# Autodesk Inventor assembly: ЛЦМК000002.00.03.00.00.00 Облегченный вариант крепления
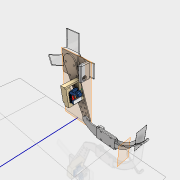
[picture p0: Inventor's stored thumbnail of the model, 180x180]
Saved by Autodesk Inventor 2021.2 (Build 252289000, 289)
## iProperties
Created: 2025-11-11
Part Number: ЛЦМК000002.00.03.00.00.00 Облегченный вариант крепления
Document SubType Name: Assembly
Designer: Захаров
Author: Захаров
## Documents named in this file (12)
- C:\Users\User\Documents\CaseARHead1\ЛЦМК000002.00.03.00.00.00 Облегченный вариант крепления.iam
- ЛЦМК000002.00.03.00.00.00 Облегченный вариант крепления.iam
- C:\Users\User\Documents\CaseARHead1\ЛЦМК000002.00.00.00.00.08-01.ipt
- C:\Users\User\Documents\CaseARHead1\ЛЦМК000002.00.00.00.00.15.ipt
- C:\Users\User\Documents\CaseARHead1\ЛЦМК000002.00.00.00.00.18-01.ipt
- C:\Users\User\Documents\CaseARHead1\ЛЦМК000002.00.00.00.00.19 мост.ipt
- C:\Users\User\Documents\CaseARHead1\ЛЦМК000002.00.00.00.00.06-10.ipt
- C:\Users\User\Documents\CaseARHead1\Сборка1.iam
- C:\Users\User\Documents\Inventor\Content Center Files\R2021\ru-RU\Screw A2 GOST 17473-80\Винт A2.M3-6gx6 ГОСТ 17473-80.ipt
- C:\Users\User\Documents\CaseARHead1\ЛЦМК000002.00.00.00.00.20 Платформа экрана.ipt
- C:\Users\User\Documents\CaseARHead1\ЛЦМК000002.00.00.00.00.13 OLED.ipt
- C:\Users\User\Documents\CaseARHead1\ЛЦМК000002.00.00.00.00.14 Фиксатор OLED.ipt
## Components (10 placed, 10 different names)
1. ЛЦМК000002.00.00.00.00.08-01:1 — Вставка:1, Вставка:2
2. ЛЦМК000002.00.00.00.00.15:1 — Вставка:1, Вставка:2, Заподлицо:1, Совмещение:1, Заподлицо:2
3. ЛЦМК000002.00.00.00.00.18-01:1 — Заподлицо:1, Совмещение:1, Заподлицо:2, Вставка:3, Вставка:4
4. ЛЦМК000002.00.00.00.00.19 мост:1 — Вставка:3, Вставка:4, Совмещение:2, Вставка:5, Заподлицо:3, Заподлицо:4
5. ЛЦМК000002.00.00.00.00.06-10:1 — Совмещение:2, Вставка:5, Совмещение:3, Совмещение:4
6. Сборка1:1 [sub-assembly] — Совмещение:3, Совмещение:4
7. Винт A2 ГОСТ 17473-80 M3-6gx6:1
8. ЛЦМК000002.00.00.00.00.20 Платформа экрана:1 — Заподлицо:3, Заподлицо:4, Вставка:6, Вставка:7, Вставка:8, Вставка:9
9. ЛЦМК000002.00.00.00.00.13 OLED:1 — Вставка:6, Вставка:7
10. ЛЦМК000002.00.00.00.00.14 Фиксатор OLED:1 — Вставка:8, Вставка:9
## Relationships (17: Insert 9, Flush 4, Mate 4)
- Вставка:1 [Insert]: ЛЦМК000002.00.00.00.00.08-01:1 ↔ ЛЦМК000002.00.00.00.00.15:1
- Вставка:2 [Insert]: ЛЦМК000002.00.00.00.00.08-01:1 ↔ ЛЦМК000002.00.00.00.00.15:1
- Заподлицо:1 [Flush]: ЛЦМК000002.00.00.00.00.15:1 ↔ ЛЦМК000002.00.00.00.00.18-01:1
- Совмещение:1 [Mate]: ЛЦМК000002.00.00.00.00.15:1 ↔ ЛЦМК000002.00.00.00.00.18-01:1
- Заподлицо:2 [Flush] (20 mm): ЛЦМК000002.00.00.00.00.15:1 ↔ ЛЦМК000002.00.00.00.00.18-01:1
- Вставка:3 [Insert]: ЛЦМК000002.00.00.00.00.18-01:1 ↔ ЛЦМК000002.00.00.00.00.19 мост:1
- Вставка:4 [Insert]: ЛЦМК000002.00.00.00.00.18-01:1 ↔ ЛЦМК000002.00.00.00.00.19 мост:1
- Совмещение:2 [Mate]: ЛЦМК000002.00.00.00.00.19 мост:1 ↔ ЛЦМК000002.00.00.00.00.06-10:1
- Вставка:5 [Insert]: ЛЦМК000002.00.00.00.00.19 мост:1 ↔ ЛЦМК000002.00.00.00.00.06-10:1
- Совмещение:3 [Mate]: ЛЦМК000002.00.00.00.00.06-10:1 ↔ Сборка1:1
- Совмещение:4 [Mate]: ЛЦМК000002.00.00.00.00.06-10:1 ↔ Сборка1:1
- Заподлицо:3 [Flush]: ЛЦМК000002.00.00.00.00.19 мост:1 ↔ ЛЦМК000002.00.00.00.00.20 Платформа экрана:1
- Заподлицо:4 [Flush]: ЛЦМК000002.00.00.00.00.19 мост:1 ↔ ЛЦМК000002.00.00.00.00.20 Платформа экрана:1
- Вставка:6 [Insert]: ЛЦМК000002.00.00.00.00.20 Платформа экрана:1 ↔ ЛЦМК000002.00.00.00.00.13 OLED:1
- Вставка:7 [Insert]: ЛЦМК000002.00.00.00.00.20 Платформа экрана:1 ↔ ЛЦМК000002.00.00.00.00.13 OLED:1
- Вставка:8 [Insert]: ЛЦМК000002.00.00.00.00.20 Платформа экрана:1 ↔ ЛЦМК000002.00.00.00.00.14 Фиксатор OLED:1
- Вставка:9 [Insert]: ЛЦМК000002.00.00.00.00.20 Платформа экрана:1 ↔ ЛЦМК000002.00.00.00.00.14 Фиксатор OLED:1
